# Autodesk Inventor assembly: 1073-2017 Launcher Assembly 2
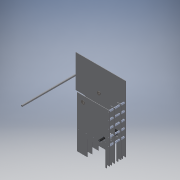
[picture p0: Inventor's stored thumbnail of the model, 180x180]
Saved by Autodesk Inventor 2016 (Build 200138000, 138)
## iProperties
Created: 2017-01-31
Part Number: 1073-2017 Launcher Assembly 2
Document SubType Name: Assembly
Designer: rasmussenf
Author: rasmussenf
## Documents named in this file (9)
- C:\Users\rasmussenf\Documents\GitHub\Robot2017\Parts\1073-2017 Launcher Assembly 2.iam
- Z:\IED\CAD\Shooter 2017\1073-2017 Shooter Inside Plate.ipt
- C:\Users\rasmussenf\Documents\GitHub\Robot2017\Parts\1,5InchChurro.ipt
- C:\Users\rasmussenf\Documents\GitHub\Robot2017\Parts\2InchChurro.ipt
- Z:\IED\CAD\Shooter 2017\1073-2017 Shooter Outside Plate Left.ipt
- C:\Users\rasmussenf\Documents\GitHub\Robot2017\VEXpro-CAD-Files-20170103\Motion\Bearings\217-3875-STEP-20140818.ipt
- C:\Users\rasmussenf\Documents\GitHub\Robot2017\VEXpro-CAD-Files-20170103\Hardware\ThunderHex\217-4002-STEP-20140806.ipt
- C:\Users\rasmussenf\Documents\GitHub\Robot2017\1073-2017 Shooter Outside Plate Right.ipt
- C:\Users\rasmussenf\Documents\GitHub\Robot2017\VEXpro-CAD-Files-20170103\Motion\Gearboxes\VersaPlanetary Gearbox\VersaPlanetary v2\v2-VersaPlanetary-1stage-with-775pro-20161031.ipt
## Components (36 placed, 8 different names)
1. 1073-2017 Shooter Outside Plate Left:1
2. 1073-2017 Shooter Inside Plate:1
3. 1,5InchChurro:1
4. 1,5InchChurro:2
5. 1,5InchChurro:3
6. 1,5InchChurro:4
7. 1,5InchChurro:5
8. 1,5InchChurro:6
9. 1,5InchChurro:7
10. 1,5InchChurro:8
11. 1,5InchChurro:9
12. 1073-2017 Shooter Inside Plate:2
13. 2InchChurro:1
14. 2InchChurro:2
15. 2InchChurro:3
16. 2InchChurro:4
17. 2InchChurro:5
18. 2InchChurro:6
19. 2InchChurro:7
20. 2InchChurro:8
21. 2InchChurro:9
22. 1073-2017 Shooter Outside Plate Left:2
23. 1,5InchChurro:10
24. 1,5InchChurro:11
25. 1,5InchChurro:12
26. 1,5InchChurro:13
27. 1,5InchChurro:14
28. 1,5InchChurro:15
29. 1,5InchChurro:16
30. 1,5InchChurro:17
31. 1,5InchChurro:18
32. 217-3875-STEP-20140818:1
33. 217-3875-STEP-20140818:2
34. 217-4002-STEP-20140806:1
35. 1073-2017 Shooter Outside Plate Right:1
36. v2-VersaPlanetary-1stage-with-775pro-20161031:1
## Relationships (70: Mate 64, Flush 6)
- [Mate]: 1073-2017 Shooter Inside Plate:1 ↔ 1,5InchChurro:1
- [Mate]: 1073-2017 Shooter Inside Plate:1 ↔ 1,5InchChurro:2
- [Mate]: 1073-2017 Shooter Inside Plate:1 ↔ 1,5InchChurro:3
- [Mate]: 1073-2017 Shooter Inside Plate:1 ↔ 1,5InchChurro:4
- [Mate]: 1073-2017 Shooter Inside Plate:1 ↔ 1,5InchChurro:5
- [Mate]: 1073-2017 Shooter Inside Plate:1 ↔ 1,5InchChurro:6
- [Mate]: 1073-2017 Shooter Inside Plate:1 ↔ 1,5InchChurro:7
- [Mate]: 1073-2017 Shooter Inside Plate:1 ↔ 1,5InchChurro:8
- [Mate]: 1073-2017 Shooter Inside Plate:1 ↔ 1,5InchChurro:9
- [Flush]: 1073-2017 Shooter Inside Plate:1 ↔ 1073-2017 Shooter Inside Plate:2
- [Flush]: 1073-2017 Shooter Inside Plate:1 ↔ 1073-2017 Shooter Inside Plate:2
- [Mate] (50.8 mm): 1073-2017 Shooter Inside Plate:1 ↔ 1073-2017 Shooter Inside Plate:2
- [Mate]: 1073-2017 Shooter Inside Plate:1 ↔ 2InchChurro:1
- [Mate]: 1073-2017 Shooter Inside Plate:2 ↔ 2InchChurro:1
- [Mate]: 1073-2017 Shooter Inside Plate:1 ↔ 2InchChurro:2
- [Mate]: 1073-2017 Shooter Inside Plate:2 ↔ 2InchChurro:2
- [Mate]: 1073-2017 Shooter Inside Plate:1 ↔ 2InchChurro:3
- [Mate]: 1073-2017 Shooter Inside Plate:2 ↔ 2InchChurro:3
- [Mate]: 1073-2017 Shooter Inside Plate:1 ↔ 2InchChurro:4
- [Mate]: 1073-2017 Shooter Inside Plate:2 ↔ 2InchChurro:4
- [Mate]: 1073-2017 Shooter Inside Plate:1 ↔ 2InchChurro:5
- [Mate]: 1073-2017 Shooter Inside Plate:2 ↔ 2InchChurro:5
- [Mate]: 1073-2017 Shooter Inside Plate:1 ↔ 2InchChurro:6
- [Mate]: 1073-2017 Shooter Inside Plate:2 ↔ 2InchChurro:6
- [Mate]: 1073-2017 Shooter Inside Plate:1 ↔ 2InchChurro:7
- [Mate]: 1073-2017 Shooter Inside Plate:2 ↔ 2InchChurro:7
- [Mate]: 1073-2017 Shooter Inside Plate:1 ↔ 2InchChurro:8
- [Mate]: 1073-2017 Shooter Inside Plate:2 ↔ 2InchChurro:8
- [Mate]: 1073-2017 Shooter Inside Plate:1 ↔ 2InchChurro:9
- [Mate]: 1073-2017 Shooter Inside Plate:2 ↔ 2InchChurro:9
- [Flush]: 1073-2017 Shooter Inside Plate:2 ↔ 1073-2017 Shooter Outside Plate Left:2
- [Flush]: 1073-2017 Shooter Inside Plate:2 ↔ 1073-2017 Shooter Outside Plate Left:2
- [Mate] (38.1 mm): 1073-2017 Shooter Inside Plate:2 ↔ 1073-2017 Shooter Outside Plate Left:2
- [Mate]: 1073-2017 Shooter Inside Plate:2 ↔ 1,5InchChurro:10
- [Mate]: 1073-2017 Shooter Outside Plate Left:2 ↔ 1,5InchChurro:10
- [Mate]: 1073-2017 Shooter Inside Plate:2 ↔ 1,5InchChurro:11
- [Mate]: 1073-2017 Shooter Outside Plate Left:2 ↔ 1,5InchChurro:11
- [Mate]: 1073-2017 Shooter Inside Plate:2 ↔ 1,5InchChurro:12
- [Mate]: 1073-2017 Shooter Outside Plate Left:2 ↔ 1,5InchChurro:12
- [Mate]: 1073-2017 Shooter Inside Plate:2 ↔ 1,5InchChurro:13
- [Mate]: 1073-2017 Shooter Outside Plate Left:2 ↔ 1,5InchChurro:13
- [Mate]: 1073-2017 Shooter Inside Plate:2 ↔ 1,5InchChurro:14
- [Mate]: 1073-2017 Shooter Outside Plate Left:2 ↔ 1,5InchChurro:14
- [Mate]: 1073-2017 Shooter Inside Plate:2 ↔ 1,5InchChurro:15
- [Mate]: 1073-2017 Shooter Outside Plate Left:2 ↔ 1,5InchChurro:15
- [Mate]: 1073-2017 Shooter Inside Plate:2 ↔ 1,5InchChurro:16
- [Mate]: 1073-2017 Shooter Outside Plate Left:2 ↔ 1,5InchChurro:16
- [Mate]: 1073-2017 Shooter Inside Plate:2 ↔ 1,5InchChurro:17
- [Mate]: 1073-2017 Shooter Outside Plate Left:2 ↔ 1,5InchChurro:17
- [Mate]: 1073-2017 Shooter Inside Plate:2 ↔ 1,5InchChurro:18
- [Mate]: 1073-2017 Shooter Outside Plate Left:2 ↔ 1,5InchChurro:18
- [Mate]: 1073-2017 Shooter Outside Plate Left:2 ↔ 217-3875-STEP-20140818:2
- [Mate]: 1073-2017 Shooter Outside Plate Left:2 ↔ 217-3875-STEP-20140818:2
- [Flush]: 1073-2017 Shooter Inside Plate:1 ↔ 1073-2017 Shooter Outside Plate Right:1
- [Flush]: 1073-2017 Shooter Inside Plate:1 ↔ 1073-2017 Shooter Outside Plate Right:1
- [Mate] (38.1 mm): 1073-2017 Shooter Inside Plate:1 ↔ 1073-2017 Shooter Outside Plate Right:1
- [Mate]: 1,5InchChurro:1 ↔ 1073-2017 Shooter Outside Plate Right:1
- [Mate]: 1,5InchChurro:2 ↔ 1073-2017 Shooter Outside Plate Right:1
- [Mate]: 1,5InchChurro:3 ↔ 1073-2017 Shooter Outside Plate Right:1
- [Mate]: 1,5InchChurro:4 ↔ 1073-2017 Shooter Outside Plate Right:1
- [Mate]: 1,5InchChurro:5 ↔ 1073-2017 Shooter Outside Plate Right:1
- [Mate]: 1,5InchChurro:6 ↔ 1073-2017 Shooter Outside Plate Right:1
- [Mate]: 1,5InchChurro:7 ↔ 1073-2017 Shooter Outside Plate Right:1
- [Mate]: 1,5InchChurro:8 ↔ 1073-2017 Shooter Outside Plate Right:1
- [Mate]: 1,5InchChurro:9 ↔ 1073-2017 Shooter Outside Plate Right:1
- [Mate]: 217-3875-STEP-20140818:1 ↔ 1073-2017 Shooter Outside Plate Right:1
- [Mate]: 217-3875-STEP-20140818:1 ↔ 1073-2017 Shooter Outside Plate Right:1
- [Mate]: 1073-2017 Shooter Outside Plate Right:1 ↔ v2-VersaPlanetary-1stage-with-775pro-20161031:1
- [Mate]: 1073-2017 Shooter Outside Plate Right:1 ↔ v2-VersaPlanetary-1stage-with-775pro-20161031:1
- [Mate]: 1073-2017 Shooter Outside Plate Right:1 ↔ v2-VersaPlanetary-1stage-with-775pro-20161031:1
## Named parameters: d70_d76 = 0 mm, d71_d77 = 0 mm, d72_d78 = 0 mm, d73_d79 = 0 mm, d74_d80 = 0 mm, d75_d87 = 0 mm, d76_d88 = 0 mm, d77_d89 = 0 mm, d78_d81 = 0 mm, d79_d82 = 0 mm, d80_d83 = 0 mm, d81_d84 = 0 mm, d82_d85 = 0 mm, d83_d86 = 0 mm
